# Autodesk Inventor assembly: Pelvis
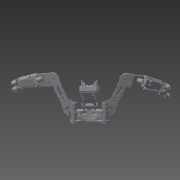
[picture p0: Inventor's stored thumbnail of the model, 180x180]
Saved by Autodesk Inventor 2018 (Build 220112000, 112)
## iProperties
Created: 2016-10-02
Part Number: Pelvis
Document SubType Name: Assembly
Designer: Val
Author: Val
## Documents named in this file (13)
- C:\Users\valer\Desktop\elysium-max-exoskeleton\src\Assemblies\Pelvis.iam
- C:\Users\valer\Desktop\elysium-max-exoskeleton\src\PelvisBaseMount.ipt
- C:\Users\valer\Desktop\elysium-max-exoskeleton\src\PelvisLink.ipt
- C:\Users\valer\Desktop\elysium-max-exoskeleton\src\PelvisMount.ipt
- C:\Users\valer\Desktop\elysium-max-exoskeleton\src\PelvisMountStem.ipt
- C:\Users\valer\Desktop\elysium-max-exoskeleton\src\PelvisSpineLink.ipt
- C:\Users\valer\Desktop\elysium-max-exoskeleton\src\PelvisSubLink.ipt
- C:\Users\valer\Desktop\elysium-max-exoskeleton\src\PelvisWingLeft.ipt
- C:\Users\valer\Desktop\elysium-max-exoskeleton\src\PelvisWingRight.ipt
- C:\Users\valer\Desktop\elysium-max-exoskeleton\src\SpineBase.ipt
- C:\Users\valer\Desktop\elysium-max-exoskeleton\src\SpacerLong.ipt
- C:\Users\valer\Desktop\elysium-max-exoskeleton\src\SpacerShort.ipt
- C:\Users\valer\Desktop\elysium-max-exoskeleton\src\BackConnector.ipt
## Components (21 placed, 12 different names)
1. PelvisBaseMount:1 — Mate:1, Mate:2, Mate:3, Mate:4, Mate:20, Mate:21, Mate:22
2. PelvisLink:1 — Mate:11, Mate:12, Mate:16, Flush:1, Mate:17
3. PelvisMount:1 — Mate:5, Mate:11, Mate:12, Mate:46, Mate:47
4. PelvisMountStem:1 — Mate:1, Mate:2, Mate:5, Mate:46, Mate:47
5. PelvisSpineLink:1 — Mate:20, Mate:21, Mate:22, Mate:27, Mate:28
6. PelvisSubLink:1 — Mate:16, Flush:1, Mate:17, Mate:25, Mate:26
7. PelvisWingLeft:1 — Mate:23, Mate:24, Mate:29, Mate:30, Mate:33, Mate:34, Mate:37, Mate:38
8. PelvisWingRight:1 — Mate:25, Mate:26, Mate:31, Mate:32, Mate:35, Mate:36, Mate:39, Mate:40
9. PelvisMountStem:2 — Mate:3, Mate:4, Mate:8, Mate:45, Angle:1
10. PelvisMount:2 — Mate:8, Mate:14, Mate:15, Mate:45, Angle:1
11. PelvisLink:2 — Mate:14, Mate:15, Mate:18, Flush:2, Mate:19
12. PelvisSubLink:2 — Mate:18, Flush:2, Mate:19, Mate:23, Mate:24
13. PelvisSpineBase:1 — Mate:27, Mate:28
14. SpacerLong:1 — Mate:29, Mate:30
15. SpacerLong:2 — Mate:31, Mate:32
16. SpacerShort:2 — Mate:33, Mate:34
17. SpacerShort:4 — Mate:35, Mate:36
18. BackConnector:1 — Mate:37, Mate:38, Mate:41, Mate:42
19. BackConnector:4 — Mate:39, Mate:40, Mate:43, Mate:44
20. SpacerShort:5 — Mate:43, Mate:44
21. SpacerShort:6 — Mate:41, Mate:42
## Relationships (45: Mate 42, Flush 2, Angle 1)
- Mate:1: PelvisBaseMount:1 ↔ PelvisMountStem:1
- Mate:2: PelvisBaseMount:1 ↔ PelvisMountStem:1
- Mate:3: PelvisBaseMount:1 ↔ PelvisMountStem:2
- Mate:4: PelvisBaseMount:1 ↔ PelvisMountStem:2
- Mate:5: PelvisMount:1 ↔ PelvisMountStem:1
- Mate:8: PelvisMountStem:2 ↔ PelvisMount:2
- Mate:11: PelvisLink:1 ↔ PelvisMount:1
- Mate:12: PelvisLink:1 ↔ PelvisMount:1
- Mate:14: PelvisMount:2 ↔ PelvisLink:2
- Mate:15: PelvisMount:2 ↔ PelvisLink:2
- Mate:16: PelvisLink:1 ↔ PelvisSubLink:1
- Flush:1: PelvisLink:1 ↔ PelvisSubLink:1
- Mate:17: PelvisLink:1 ↔ PelvisSubLink:1
- Mate:18: PelvisLink:2 ↔ PelvisSubLink:2
- Flush:2: PelvisLink:2 ↔ PelvisSubLink:2
- Mate:19: PelvisLink:2 ↔ PelvisSubLink:2
- Mate:20: PelvisBaseMount:1 ↔ PelvisSpineLink:1
- Mate:21: PelvisBaseMount:1 ↔ PelvisSpineLink:1
- Mate:22: PelvisBaseMount:1 ↔ PelvisSpineLink:1
- Mate:23: PelvisWingLeft:1 ↔ PelvisSubLink:2
- Mate:24: PelvisWingLeft:1 ↔ PelvisSubLink:2
- Mate:25: PelvisSubLink:1 ↔ PelvisWingRight:1
- Mate:26: PelvisSubLink:1 ↔ PelvisWingRight:1
- Mate:27: PelvisSpineLink:1 ↔ PelvisSpineBase:1
- Mate:28: PelvisSpineLink:1 ↔ PelvisSpineBase:1
- Mate:29: PelvisWingLeft:1 ↔ SpacerLong:1
- Mate:30: PelvisWingLeft:1 ↔ SpacerLong:1
- Mate:31: PelvisWingRight:1 ↔ SpacerLong:2
- Mate:32: PelvisWingRight:1 ↔ SpacerLong:2
- Mate:33: PelvisWingLeft:1 ↔ SpacerShort:2
- Mate:34: PelvisWingLeft:1 ↔ SpacerShort:2
- Mate:35: PelvisWingRight:1 ↔ SpacerShort:4
- Mate:36: PelvisWingRight:1 ↔ SpacerShort:4
- Mate:37: PelvisWingLeft:1 ↔ BackConnector:1
- Mate:38: PelvisWingLeft:1 ↔ BackConnector:1
- Mate:39: PelvisWingRight:1 ↔ BackConnector:4
- Mate:40: PelvisWingRight:1 ↔ BackConnector:4
- Mate:41: BackConnector:1 ↔ SpacerShort:6
- Mate:42: BackConnector:1 ↔ SpacerShort:6
- Mate:43: BackConnector:4 ↔ SpacerShort:5
- Mate:44: BackConnector:4 ↔ SpacerShort:5
- Mate:45: PelvisMountStem:2 ↔ PelvisMount:2
- Angle:1 (180 deg): PelvisMountStem:2 ↔ PelvisMount:2
- Mate:46: PelvisMount:1 ↔ PelvisMountStem:1
- Mate:47: PelvisMount:1 ↔ PelvisMountStem:1
